# Autodesk Inventor assembly: Caufield_Engine_Assembly
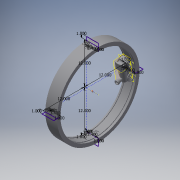
[picture p0: Inventor's stored thumbnail of the model, 180x180]
Saved by Autodesk Inventor 2016 (Build 200138000, 138)
## iProperties
Created: 2018-01-17
Part Number: Caufield_Engine_Assembly
Document SubType Name: Assembly
Designer: The Panda
Author: The Panda
## Documents named in this file (12)
- E:\IED7_CaufieldE\IED7_Caufield_P4.1_Toy_Train\Caufield_TrainOnLOOPTrack.iam
- E:\IED7_CaufieldE\IED7_Caufield_P4.1_Toy_Train\Caufield_Engine_Body.ipt
- E:\IED7_CaufieldE\IED7_Caufield_P4.1_Toy_Train\Caufield_Stack.ipt
- E:\IED7_CaufieldE\IED7_Caufield_P4.1_Toy_Train\Caufield_Hitch_Magnet.ipt
- E:\IED7_CaufieldE\IED7_Caufield_P4.1_Toy_Train\Caufield_Hitch_Peg.ipt
- E:\IED7_CaufieldE\IED7_Caufield_P4.1_Toy_Train\Caufield_Cow_Catcher.ipt
- E:\IED7_CaufieldE\IED7_Caufield_P4.1_Toy_Train\Caufield_Wheel.ipt
- E:\IED7_CaufieldE\IED7_Caufield_P4.1_Toy_Train\Caufield_Axle_Peg.ipt
- E:\IED7_CaufieldE\IED7_Caufield_P4.1_Toy_Train\Caufield_Linkage_Arm.ipt
- E:\IED7_CaufieldE\IED7_Caufield_P4.1_Toy_Train\Caufield_Linkage_Peg.ipt
- E:\IED7_CaufieldE\IED7_Caufield_P4.1_Toy_Train\Caufield_LOOP_Track.ipt
- E:\IED7_CaufieldE\IED7_Caufield_P4.1_Toy_Train\P4_1PivotCube.ipt
## Components (24 placed, 12 different names)
1. Caufield_Engine_Body:1 — Insert:1, Angle:1, Mate:1, Mate:2, Insert:3, Insert:4, Angle:6, Insert:5, Insert:6, Insert:7, Insert:8, Angle:7, Angle:8, DriveAngle, Mate:5, Mate:6, Flush:2
2. Caufield_Stack:1 — Insert:1, Angle:1
3. Caufield_Hitch_Magnet:1 — Mate:1, Mate:2, Insert:2
4. Caufield_Hitch_Peg:1 — Insert:2, Angle:6
5. Caufield_Cow_Catcher:1 — Insert:3, Insert:4
6. Caufield_Wheel:1drive wheel — Insert:6, Insert:10, Insert:15, Insert:17, DriveAngle, Angle:12, Angle:16
7. Caufield_Wheel:2 — Insert:7, Insert:11, Insert:14, Insert:19, Angle:9, Angle:14, Angle:17
8. Caufield_Wheel:3 — Insert:8, Insert:12, Insert:13, Insert:20, Angle:13, Angle:18
9. Caufield_Wheel:4 — Insert:5, Insert:9, Insert:16, Insert:18, Angle:9, Angle:11, Angle:15
10. Caufield_Linkage_Peg:1 — Insert:17, Angle:12
11. Caufield_Linkage_Peg:2 — Insert:18, Angle:11
12. Caufield_Linkage_Peg:3 — Insert:19, Angle:14
13. Caufield_Linkage_Peg:4 — Insert:20, Angle:13
14. Caufield_Linkage_Arm:1 — Insert:13, Insert:14, Angle:7
15. Caufield_Linkage_Arm:2 — Insert:15, Insert:16, Angle:8
16. Caufield_Axle_Peg:1 — Insert:12, Angle:18
17. Caufield_Axle_Peg:2 — Insert:11, Angle:17
18. Caufield_Axle_Peg:3 — Insert:10, Angle:16
19. Caufield_Axle_Peg:4 — Insert:9, Angle:15
20. P4_1PivotCube:1 — Mate:4, Mate:5, Mate:6
21. Caufield_LOOP_Track:1
22. Caufield_LOOP_Track:5
23. Caufield_LOOP_Track:3
24. Caufield_LOOP_Track:4 — Mate:3, Flush:2
## Component patterns: (4 elements, first: Caufield_LOOP_Track:1)
## Relationships (41: Insert 20, Angle 14, Mate 6, Flush 1)
- Insert:1: Caufield_Engine_Body:1 ↔ Caufield_Stack:1
- Angle:1 (0 deg): Caufield_Engine_Body:1 ↔ Caufield_Stack:1
- Mate:1: Caufield_Engine_Body:1 ↔ Caufield_Hitch_Magnet:1
- Mate:2: Caufield_Engine_Body:1 ↔ Caufield_Hitch_Magnet:1
- Insert:2: Caufield_Hitch_Magnet:1 ↔ Caufield_Hitch_Peg:1
- Insert:3: Caufield_Engine_Body:1 ↔ Caufield_Cow_Catcher:1
- Insert:4: Caufield_Engine_Body:1 ↔ Caufield_Cow_Catcher:1
- Angle:6 (0 deg): Caufield_Engine_Body:1 ↔ Caufield_Hitch_Peg:1
- Insert:5 (0.0254 mm): Caufield_Engine_Body:1 ↔ Caufield_Wheel:4
- Insert:6 (0.0254 mm): Caufield_Engine_Body:1 ↔ Caufield_Wheel:1drive wheel
- Insert:7 (0.0254 mm): Caufield_Engine_Body:1 ↔ Caufield_Wheel:2
- Insert:8 (0.0254 mm): Caufield_Engine_Body:1 ↔ Caufield_Wheel:3
- Insert:9 (0.0254 mm): Caufield_Wheel:4 ↔ Caufield_Axle_Peg:4
- Insert:10 (0.0254 mm): Caufield_Wheel:1drive wheel ↔ Caufield_Axle_Peg:3
- Insert:11 (0.0254 mm): Caufield_Wheel:2 ↔ Caufield_Axle_Peg:2
- Insert:12 (0.0254 mm): Caufield_Wheel:3 ↔ Caufield_Axle_Peg:1
- Insert:13 (0.0254 mm): Caufield_Wheel:3 ↔ Caufield_Linkage_Arm:1
- Insert:14 (0.0254 mm): Caufield_Wheel:2 ↔ Caufield_Linkage_Arm:1
- Insert:15 (0.0254 mm): Caufield_Wheel:1drive wheel ↔ Caufield_Linkage_Arm:2
- Insert:16 (0.0254 mm): Caufield_Wheel:4 ↔ Caufield_Linkage_Arm:2
- Insert:17 (0.0254 mm): Caufield_Wheel:1drive wheel ↔ Caufield_Linkage_Peg:1
- Insert:18 (0.0254 mm): Caufield_Wheel:4 ↔ Caufield_Linkage_Peg:2
- Insert:19: Caufield_Wheel:2 ↔ Caufield_Linkage_Peg:3
- Insert:20 (0.0254 mm): Caufield_Wheel:3 ↔ Caufield_Linkage_Peg:4
- Angle:7 (0 deg): Caufield_Engine_Body:1 ↔ Caufield_Linkage_Arm:1
- Angle:8 (0 deg): Caufield_Engine_Body:1 ↔ Caufield_Linkage_Arm:2
- Angle:9 (180 deg): Caufield_Wheel:2 ↔ Caufield_Wheel:4
- DriveAngle [Angle] (-3682.8 deg): Caufield_Engine_Body:1 ↔ Caufield_Wheel:1drive wheel
- Angle:11 (0 deg): Caufield_Wheel:4 ↔ Caufield_Linkage_Peg:2
- Angle:12 (0 deg): Caufield_Wheel:1drive wheel ↔ Caufield_Linkage_Peg:1
- Angle:13 (0 deg): Caufield_Wheel:3 ↔ Caufield_Linkage_Peg:4
- Angle:14 (0 deg): Caufield_Wheel:2 ↔ Caufield_Linkage_Peg:3
- Angle:15 (0 deg): Caufield_Wheel:4 ↔ Caufield_Axle_Peg:4
- Angle:16 (0 deg): Caufield_Wheel:1drive wheel ↔ Caufield_Axle_Peg:3
- Angle:17 (0 deg): Caufield_Wheel:2 ↔ Caufield_Axle_Peg:2
- Angle:18 (0 deg): Caufield_Wheel:3 ↔ Caufield_Axle_Peg:1
- Mate:3: Caufield_LOOP_Track:4
- Mate:4: P4_1PivotCube:1
- Mate:5 (259.842 mm): Caufield_Engine_Body:1 ↔ P4_1PivotCube:1
- Mate:6 (-63.5 mm): Caufield_Engine_Body:1 ↔ P4_1PivotCube:1
- Flush:2 (17.78 mm): Caufield_Engine_Body:1 ↔ Caufield_LOOP_Track:4
## Named parameters: Angle = -3682.8 deg, Angle2 = 360 deg
